# Autodesk Inventor assembly: EvelShortMidFrame
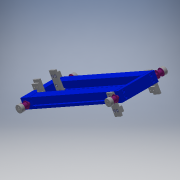
[picture p0: Inventor's stored thumbnail of the model, 180x180]
Saved by Autodesk Inventor 2019 (Build 230136000, 136)
## iProperties
Created: 2019-09-29
Part Number: EvelShortMidFrame
Document SubType Name: Assembly
Designer: james
Author: james
## Documents named in this file (5)
- F:\JimsDesign\Jims2020FTC\EvelShortMidFrame.iam
- F:\JimsDesign\Jims2020FTC\FullElevatorShart.iam
- F:\JimsDesign\Jims2020FTC\SliderLeft.iam
- F:\JimsDesign\Jims2020FTC\SliderRight.iam
- F:\JimsDesign\Jims2020FTC\ShortElevatorFrame.iam
## Components (7 placed, 4 different names)
1. ShortElevatorFrame:1 [sub-assembly] — Mate:2, Mate:17, Mate:18, Mate:19, Mate:20, Mate:21, Mate:22, Mate:23, Mate:24, Mate:25, Mate:26, Mate:27, Mate:28, Mate:29, Mate:30, Mate:31
2. FullElevatorShart:1 [sub-assembly] — Mate:17, Mate:19
3. FullElevatorShart:2 [sub-assembly] — Mate:2, Mate:18
4. SliderRight:1 [sub-assembly] — Mate:20, Mate:21, Mate:22
5. SliderRight:3 [sub-assembly] — Mate:29, Mate:30, Mate:31
6. SliderLeft:1 [sub-assembly] — Mate:23, Mate:24, Mate:25
7. SliderLeft:2 [sub-assembly] — Mate:26, Mate:27, Mate:28
## Relationships (16: Mate 16)
- Mate:2: ShortElevatorFrame:1 ↔ FullElevatorShart:2
- Mate:17: ShortElevatorFrame:1 ↔ FullElevatorShart:1
- Mate:18: ShortElevatorFrame:1 ↔ FullElevatorShart:2
- Mate:19: ShortElevatorFrame:1 ↔ FullElevatorShart:1
- Mate:20: ShortElevatorFrame:1 ↔ SliderRight:1
- Mate:21: ShortElevatorFrame:1 ↔ SliderRight:1
- Mate:22: ShortElevatorFrame:1 ↔ SliderRight:1
- Mate:23: ShortElevatorFrame:1 ↔ SliderLeft:1
- Mate:24: ShortElevatorFrame:1 ↔ SliderLeft:1
- Mate:25: ShortElevatorFrame:1 ↔ SliderLeft:1
- Mate:26: ShortElevatorFrame:1 ↔ SliderLeft:2
- Mate:27: ShortElevatorFrame:1 ↔ SliderLeft:2
- Mate:28: ShortElevatorFrame:1 ↔ SliderLeft:2
- Mate:29: ShortElevatorFrame:1 ↔ SliderRight:3
- Mate:30: ShortElevatorFrame:1 ↔ SliderRight:3
- Mate:31: ShortElevatorFrame:1 ↔ SliderRight:3
